# Autodesk Inventor assembly: god only calls me a mistake because he recognizes i will be his end
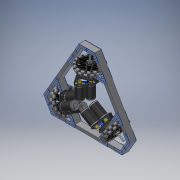
[picture p0: Inventor's stored thumbnail of the model, 180x180]
Saved by Autodesk Inventor 2018 (Build 220112000, 112)
## iProperties
Created: 2020-03-24
Part Number: god only calls me a mistake because he recognizes i will be his end
Document SubType Name: Assembly
Designer: maste
Author: maste
## Documents named in this file (6)
- C:\Users\maste\OneDrive\Documents\GitHub\2020CAD (offseason)\The Chad Kiwi\Main Assembly File\god only calls me a mistake because he recognizes i will be his end.iam
- C:\Users\maste\OneDrive\Documents\GitHub\2020CAD (offseason)\The Chad Kiwi\Part Files\Frame.ipt
- C:\Users\maste\OneDrive\Documents\GitHub\2020CAD (offseason)\The Chad Kiwi\Part Files\gearbox\WCP_SS_-_Single_Speed_Base_Kit_217-3421.iam
- C:\Users\maste\OneDrive\Documents\GitHub\2020CAD (offseason)\The Chad Kiwi\Part Files\8_Omni-Directional_Wheel_217-2613.iam
- C:\Users\maste\OneDrive\Documents\GitHub\2020CAD (offseason)\The Chad Kiwi\Part Files\60 gusset.ipt
- C:\Users\maste\OneDrive\Documents\GitHub\2020CAD (offseason)\The Chad Kiwi\Part Files\120 gusset.ipt
## Components (31 placed, 5 different names)
1. Frame:1 — Mate:1, Mate:2, Mate:3, Mate:4, Mate:5, Mate:6, Mate:7, Mate:8, Mate:9, Mate:10, Mate:11, Mate:12, Mate:13, Mate:14, Mate:15, Mate:16, Flush:1, Flush:2, Mate:17, Flush:3, Flush:4, Mate:18, Mate:19, Mate:20, Mate:21, Mate:22, Mate:23, Mate:24, Mate:25, Mate:26, Mate:27, Flush:5, Flush:6, Flush:7, Flush:8, Flush:9, Flush:10, Flush:11, Flush:12, Flush:13, Flush:14, Flush:15, Flush:16, Flush:17, Flush:18, Flush:19, Flush:20, Flush:21, Flush:22, Flush:23, Flush:24, Mate:28, Mate:29, Mate:30, Mate:31, Mate:32, Mate:33, Mate:34, Mate:35, Mate:36, Mate:37, Mate:38, Mate:39, Flush:25, Flush:26, Flush:27, Flush:28, Flush:29, Flush:30, Flush:31, Flush:32, Flush:33, Flush:34, Flush:35, Flush:36, Flush:37, Flush:38, Flush:39, Flush:40, Flush:41, Flush:42, Flush:43, Flush:44, Flush:45, Flush:46, Flush:47, Flush:48
2. WCP_SS_-_Single_Speed_Base_Kit_217-3421:1 [sub-assembly] — Mate:1, Mate:2, Mate:3
3. WCP_SS_-_Single_Speed_Base_Kit_217-3421:2 [sub-assembly] — Mate:5, Mate:8, Mate:9
4. WCP_SS_-_Single_Speed_Base_Kit_217-3421:3 [sub-assembly] — Mate:4, Mate:6, Mate:7
5. 8_Omni-Directional_Wheel_217-2613:1 [sub-assembly] — Mate:12, Mate:14
6. 8_Omni-Directional_Wheel_217-2613:2 [sub-assembly] — Mate:11, Mate:15
7. 8_Omni-Directional_Wheel_217-2613:3 [sub-assembly] — Mate:10, Mate:13
8. 60 gusset:1 — Mate:24, Flush:21, Flush:24
9. 60 gusset:2 — Mate:18, Flush:9, Flush:12
10. 60 gusset:3 — Mate:27, Flush:5, Flush:8
11. 60 gusset:4 — Mate:20, Flush:14, Flush:16
12. 60 gusset:5 — Mate:16, Flush:1, Flush:2
13. 60 gusset:6 — Mate:22, Flush:17, Flush:19
14. 60 gusset:7 — Mate:23, Flush:18, Flush:20
15. 60 gusset:8 — Mate:25, Flush:22, Flush:23
16. 60 gusset:9 — Mate:19, Flush:10, Flush:11
17. 60 gusset:10 — Mate:26, Flush:6, Flush:7
18. 60 gusset:11 — Mate:21, Flush:13, Flush:15
19. 60 gusset:12 — Mate:17, Flush:3, Flush:4
20. 120 gusset:1 — Mate:36, Flush:34, Flush:36
21. 120 gusset:2 — Mate:37, Flush:33, Flush:35
22. 120 gusset:3 — Mate:34, Flush:29, Flush:31
23. 120 gusset:4 — Mate:35, Flush:30, Flush:32
24. 120 gusset:5 — Mate:32, Flush:25, Flush:28
25. 120 gusset:6 — Mate:33, Flush:26, Flush:27
26. 120 gusset:7 — Mate:30, Flush:41, Flush:44
27. 120 gusset:8 — Mate:31, Flush:42, Flush:43
28. 120 gusset:9 — Mate:29, Flush:45, Flush:48
29. 120 gusset:10 — Mate:28, Flush:46, Flush:47
30. 120 gusset:11 — Mate:38, Flush:38, Flush:39
31. 120 gusset:12 — Mate:39, Flush:37, Flush:40
## Relationships (87: Flush 48, Mate 39)
- Mate:1: Frame:1 ↔ WCP_SS_-_Single_Speed_Base_Kit_217-3421:1
- Mate:2: Frame:1 ↔ WCP_SS_-_Single_Speed_Base_Kit_217-3421:1
- Mate:3: Frame:1 ↔ WCP_SS_-_Single_Speed_Base_Kit_217-3421:1
- Mate:4: Frame:1 ↔ WCP_SS_-_Single_Speed_Base_Kit_217-3421:3
- Mate:5: Frame:1 ↔ WCP_SS_-_Single_Speed_Base_Kit_217-3421:2
- Mate:6: Frame:1 ↔ WCP_SS_-_Single_Speed_Base_Kit_217-3421:3
- Mate:7: Frame:1 ↔ WCP_SS_-_Single_Speed_Base_Kit_217-3421:3
- Mate:8: Frame:1 ↔ WCP_SS_-_Single_Speed_Base_Kit_217-3421:2
- Mate:9: Frame:1 ↔ WCP_SS_-_Single_Speed_Base_Kit_217-3421:2
- Mate:10: Frame:1 ↔ 8_Omni-Directional_Wheel_217-2613:3
- Mate:11: Frame:1 ↔ 8_Omni-Directional_Wheel_217-2613:2
- Mate:12: Frame:1 ↔ 8_Omni-Directional_Wheel_217-2613:1
- Mate:13: Frame:1 ↔ 8_Omni-Directional_Wheel_217-2613:3
- Mate:14: Frame:1 ↔ 8_Omni-Directional_Wheel_217-2613:1
- Mate:15: Frame:1 ↔ 8_Omni-Directional_Wheel_217-2613:2
- Mate:16: Frame:1 ↔ 60 gusset:5
- Flush:1: Frame:1 ↔ 60 gusset:5
- Flush:2: Frame:1 ↔ 60 gusset:5
- Mate:17: Frame:1 ↔ 60 gusset:12
- Flush:3: Frame:1 ↔ 60 gusset:12
- Flush:4: Frame:1 ↔ 60 gusset:12
- Mate:18: Frame:1 ↔ 60 gusset:2
- Mate:19: Frame:1 ↔ 60 gusset:9
- Mate:20: Frame:1 ↔ 60 gusset:4
- Mate:21: Frame:1 ↔ 60 gusset:11
- Mate:22: Frame:1 ↔ 60 gusset:6
- Mate:23: Frame:1 ↔ 60 gusset:7
- Mate:24: Frame:1 ↔ 60 gusset:1
- Mate:25: Frame:1 ↔ 60 gusset:8
- Mate:26: Frame:1 ↔ 60 gusset:10
- Mate:27: Frame:1 ↔ 60 gusset:3
- Flush:5: Frame:1 ↔ 60 gusset:3
- Flush:6: Frame:1 ↔ 60 gusset:10
- Flush:7: Frame:1 ↔ 60 gusset:10
- Flush:8: Frame:1 ↔ 60 gusset:3
- Flush:9: Frame:1 ↔ 60 gusset:2
- Flush:10: Frame:1 ↔ 60 gusset:9
- Flush:11: Frame:1 ↔ 60 gusset:9
- Flush:12: Frame:1 ↔ 60 gusset:2
- Flush:13: Frame:1 ↔ 60 gusset:11
- Flush:14: Frame:1 ↔ 60 gusset:4
- Flush:15: Frame:1 ↔ 60 gusset:11
- Flush:16: Frame:1 ↔ 60 gusset:4
- Flush:17: Frame:1 ↔ 60 gusset:6
- Flush:18: Frame:1 ↔ 60 gusset:7
- Flush:19: Frame:1 ↔ 60 gusset:6
- Flush:20: Frame:1 ↔ 60 gusset:7
- Flush:21: Frame:1 ↔ 60 gusset:1
- Flush:22: Frame:1 ↔ 60 gusset:8
- Flush:23: Frame:1 ↔ 60 gusset:8
- Flush:24: Frame:1 ↔ 60 gusset:1
- Mate:28: Frame:1 ↔ 120 gusset:10
- Mate:29: Frame:1 ↔ 120 gusset:9
- Mate:30: Frame:1 ↔ 120 gusset:7
- Mate:31: Frame:1 ↔ 120 gusset:8
- Mate:32: Frame:1 ↔ 120 gusset:5
- Mate:33: Frame:1 ↔ 120 gusset:6
- Mate:34: Frame:1 ↔ 120 gusset:3
- Mate:35: Frame:1 ↔ 120 gusset:4
- Mate:36: Frame:1 ↔ 120 gusset:1
- Mate:37: Frame:1 ↔ 120 gusset:2
- Mate:38: Frame:1 ↔ 120 gusset:11
- Mate:39: Frame:1 ↔ 120 gusset:12
- Flush:25: Frame:1 ↔ 120 gusset:5
- Flush:26: Frame:1 ↔ 120 gusset:6
- Flush:27: Frame:1 ↔ 120 gusset:6
- Flush:28: Frame:1 ↔ 120 gusset:5
- Flush:29: Frame:1 ↔ 120 gusset:3
- Flush:30: Frame:1 ↔ 120 gusset:4
- Flush:31: Frame:1 ↔ 120 gusset:3
- Flush:32: Frame:1 ↔ 120 gusset:4
- Flush:33: Frame:1 ↔ 120 gusset:2
- Flush:34: Frame:1 ↔ 120 gusset:1
- Flush:35: Frame:1 ↔ 120 gusset:2
- Flush:36: Frame:1 ↔ 120 gusset:1
- Flush:37: Frame:1 ↔ 120 gusset:12
- Flush:38: Frame:1 ↔ 120 gusset:11
- Flush:39: Frame:1 ↔ 120 gusset:11
- Flush:40: Frame:1 ↔ 120 gusset:12
- Flush:41: Frame:1 ↔ 120 gusset:7
- Flush:42: Frame:1 ↔ 120 gusset:8
- Flush:43: Frame:1 ↔ 120 gusset:8
- Flush:44: Frame:1 ↔ 120 gusset:7
- Flush:45: Frame:1 ↔ 120 gusset:9
- Flush:46: Frame:1 ↔ 120 gusset:10
- Flush:47: Frame:1 ↔ 120 gusset:10
- Flush:48: Frame:1 ↔ 120 gusset:9
